# Autodesk Inventor assembly: Assembly2
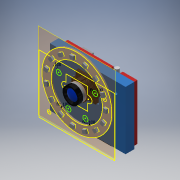
[picture p0: Inventor's stored thumbnail of the model, 180x180]
Saved by Autodesk Inventor 2017 (Build 210142000, 142)
## iProperties
Created: 2016-12-20
Part Number: Assembly2
Document SubType Name: Assembly
Designer: PLTW
Author: PLTW
## Documents named in this file (7)
- C:\Users\PLTW\Documents\Inventor\PixyCam and Gimbal\Assembly2.iam
- C:\Users\PLTW\Documents\Inventor\PixyCam and Gimbal\PixyCamKinda.ipt
- C:\Users\PLTW\Documents\Inventor\PixyCam and Gimbal\focusSpacer.ipt
- C:\Users\PLTW\Documents\Inventor\PixyCam and Gimbal\LEDRing.ipt
- C:\Users\PLTW\Documents\Inventor\PixyCam and Gimbal\backCase.ipt
- C:\Users\PLTW\Documents\Inventor\PixyCam and Gimbal\frontCase.ipt
- C:\Users\PLTW\Documents\Inventor\PixyCam and Gimbal\Ring Front.ipt
## Components (6 placed, 6 different names)
1. PixyCamKinda:1 — Insert:1, Insert:2, Flush:1, Flush:2, Flush:3, Flush:4
2. focusSpacer:1 — Insert:1
3. LEDRing:1 — Insert:2, Flush:6, Flush:7
4. backCase:1 — Flush:1, Flush:2, Flush:5
5. frontCase:1 — Flush:3, Flush:4, Flush:5
6. Ring Front:1 — Flush:6, Flush:7
## Relationships (9: Flush 7, Insert 2)
- Insert:1: PixyCamKinda:1 ↔ focusSpacer:1
- Insert:2: PixyCamKinda:1 ↔ LEDRing:1
- Flush:1: PixyCamKinda:1 ↔ backCase:1
- Flush:2: PixyCamKinda:1 ↔ backCase:1
- Flush:3: PixyCamKinda:1 ↔ frontCase:1
- Flush:4: PixyCamKinda:1 ↔ frontCase:1
- Flush:5: backCase:1 ↔ frontCase:1
- Flush:6: LEDRing:1 ↔ Ring Front:1
- Flush:7: LEDRing:1 ↔ Ring Front:1
